# Autodesk Inventor assembly: gripperBracketAssembly
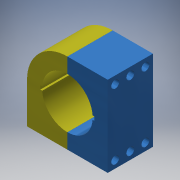
[picture p0: Inventor's stored thumbnail of the model, 180x180]
Saved by Autodesk Inventor 2018.2 (Build 222227000, 227)
## iProperties
Created: 2018-02-13
Part Number: gripperBracketAssembly
Document SubType Name: Assembly
Designer: steele
Author: steele
## Documents named in this file (3)
- D:\snobotics\CAD-Development\robSteele\2018-FRC\Gripper\gripperBracketAssembly.iam
- D:\snobotics\CAD-Development\robSteele\2018-FRC\Gripper\gripperBracketA.ipt
- D:\snobotics\CAD-Development\robSteele\2018-FRC\Gripper\gripperBracketB.ipt
## Components (2 placed, 2 different names)
1. gripperBracketA:1 — Mate:1, Mate:2, Mate:3, Flush:1
2. gripperBracketB:1 — Mate:1, Mate:2, Mate:3
## Relationships (4: Mate 3, Flush 1)
- Mate:1: gripperBracketA:1 ↔ gripperBracketB:1
- Mate:2: gripperBracketA:1 ↔ gripperBracketB:1
- Mate:3: gripperBracketA:1 ↔ gripperBracketB:1
- Flush:1 (-9.525 mm): gripperBracketA:1
